# Autodesk Inventor assembly: StereoPi
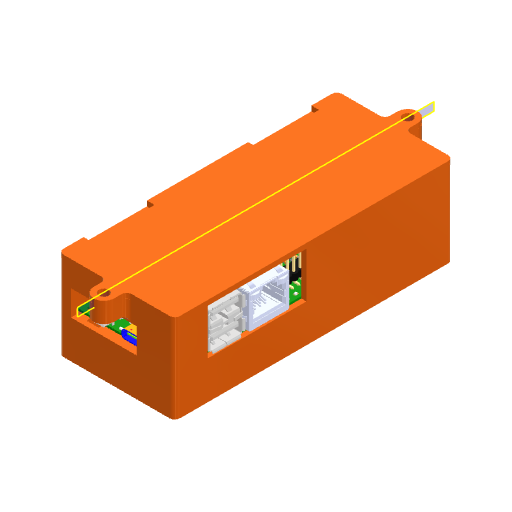
[picture p0: Inventor's stored thumbnail of the model, 512x512]
Saved by Autodesk Inventor 2025.2 (Build 292293000, 293)
## iProperties
Created: 2025-03-12
Part Number: StereoPi
Document SubType Name: Assembly
Designer: rolan
Author: rolan
## Documents named in this file (4)
- C:\Users\rolan\Documents\PhD\Inventor\Assembly\StereoPi.iam
- C:\Users\rolan\Documents\PhD\Inventor\Parts\StereoPiBracket.ipt
- C:\Users\rolan\Documents\PhD\Inventor\Parts\StereoPiBracketLid.ipt
- C:\Users\rolan\Documents\PhD\Inventor\3D Files\stereopi_v2\stereopi_v2\stereopi_v2.ipt
## Components (3 placed, 3 different names)
1. StereoPiBracket:1 — Mate:1, Mate:2, Mate:3, Mate:4, Mate:5
2. StereoPiBracketLid:1 — Mate:1, Mate:2, Mate:3
3. stereopi_v2:1 — Mate:4, Mate:5
## Relationships (5: Mate 5)
- Mate:1: StereoPiBracket:1 ↔ StereoPiBracketLid:1
- Mate:2: StereoPiBracket:1 ↔ StereoPiBracketLid:1
- Mate:3: StereoPiBracket:1 ↔ StereoPiBracketLid:1
- Mate:4: StereoPiBracket:1 ↔ stereopi_v2:1
- Mate:5: StereoPiBracket:1 ↔ stereopi_v2:1
